# Autodesk Inventor assembly: inchHexSocketHanger
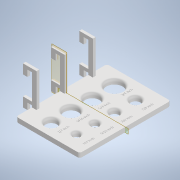
[picture p0: Inventor's stored thumbnail of the model, 180x180]
Saved by Autodesk Inventor 2020.2 (Build 242310000, 310)
## iProperties
Created: 2020-03-17
Part Number: inchHexSocketHanger
Document SubType Name: Assembly
Designer: robst
Author: robst
## Documents named in this file (3)
- C:\git\CAD-Development\robSteele\HouseProjects\Garage\Ikea\inchHexSocketHanger.iam
- C:\git\CAD-Development\robSteele\HouseProjects\Garage\Ikea\threeStartConfigurationV01.ipt
- C:\git\CAD-Development\robSteele\HouseProjects\Garage\Ikea\inchHexSocketSetOf8.ipt
## Components (2 placed, 2 different names)
1. threeStartConfigurationV01:1 — Mate:1, Flush:1, Flush:2
2. inchHexSocketSetOf8:1 — Mate:1, Flush:1, Flush:2
## Relationships (3: Flush 2, Mate 1)
- Mate:1: threeStartConfigurationV01:1 ↔ inchHexSocketSetOf8:1
- Flush:1: threeStartConfigurationV01:1 ↔ inchHexSocketSetOf8:1
- Flush:2: threeStartConfigurationV01:1 ↔ inchHexSocketSetOf8:1
